# Autodesk Inventor assembly: Temp_controller_demo_ASSY
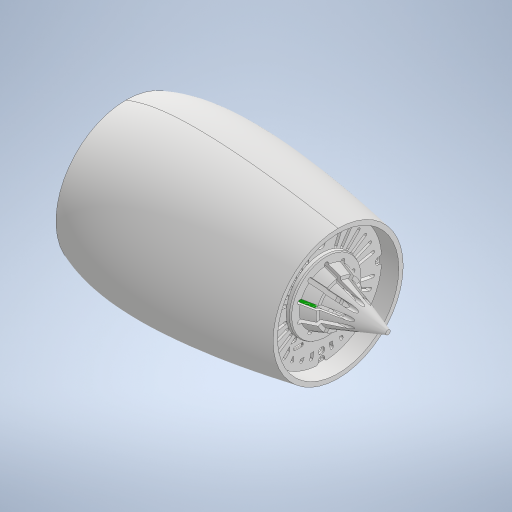
[picture p0: Inventor's stored thumbnail of the model, 512x512]
Saved by Autodesk Inventor 2024 (Build 280153000, 153)
## iProperties
Created: 2026-04-14
Part Number: Temp_controller_demo_ASSY
Document SubType Name: Assembly
Designer: Péter
Author: Péter
## Documents named in this file (5)
- D:\Inventor\Repositories\Temperature-Controller\Temp_controller_demo_ASSY.iam
- D:\Inventor\Repositories\Temperature-Controller\Import\Altium\Rack Temperature & Fan Controller_Step_Rev.1.0._2026-04-14\Rack Temperature & Fan Controller_Step_Rev.1.0._2026-04-14.ipt
- D:\Inventor\Repositories\Temperature-Controller\Temp_controller_trent.ipt
- D:\Inventor\Repositories\Temperature-Controller\Temp_controller_trent_back.ipt
- D:\Inventor\Repositories\Temperature-Controller\Import\CNPS8900\CNPS8900.ipt
## Components (4 placed, 4 different names)
1. Rack Temperature & Fan Controller_Step_Rev.1.0._2026-04-14:1 — Insert:1, Insert:2, Insert:3, Insert:4
2. Temp_controller_trent:1 — Insert:5, Insert:6, Insert:7
3. Temp_controller_trent_back:1 — Insert:1, Insert:2, Insert:3, Insert:4, Insert:5, Insert:6
4. CNPS8900:1 — Insert:7
## Relationships (7: Insert 7)
- Insert:1: Rack Temperature & Fan Controller_Step_Rev.1.0._2026-04-14:1 ↔ Temp_controller_trent_back:1
- Insert:2: Rack Temperature & Fan Controller_Step_Rev.1.0._2026-04-14:1 ↔ Temp_controller_trent_back:1
- Insert:3: Rack Temperature & Fan Controller_Step_Rev.1.0._2026-04-14:1 ↔ Temp_controller_trent_back:1
- Insert:4: Rack Temperature & Fan Controller_Step_Rev.1.0._2026-04-14:1 ↔ Temp_controller_trent_back:1
- Insert:5: Temp_controller_trent:1 ↔ Temp_controller_trent_back:1
- Insert:6: Temp_controller_trent:1 ↔ Temp_controller_trent_back:1
- Insert:7: Temp_controller_trent:1 ↔ CNPS8900:1
